# Autodesk Inventor assembly: tacho
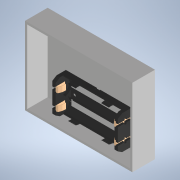
[picture p0: Inventor's stored thumbnail of the model, 180x180]
Saved by Autodesk Inventor 2022 (Build 260153000, 153)
## iProperties
Created: 2024-07-12
Part Number: tacho
Document SubType Name: Assembly
Designer: Капустяник Андрей
Author: Капустяник Андрей
## Documents named in this file (5)
- C:\Users\akapu\OneDrive\Документы\Git\camp2024\tacho_case\tacho.iam
- C:\Users\akapu\OneDrive\Документы\Git\camp2024\tacho_case\tacho_base.ipt
- C:\Users\akapu\OneDrive\Документы\Git\camp2024\tacho_case\WEH000802ALPP5N00000.ipt
- C:\Users\akapu\OneDrive\Документы\Git\camp2024\tacho_case\Hold_18650-2p_smd.ipt
- C:\Users\akapu\OneDrive\Документы\Git\camp2024\tacho_case\tacho_board.ipt
## Components (4 placed, 4 different names)
1. tacho_base:1 — Совмещение:3, Совмещение:4, Заподлицо:1, Совмещение:5, Совмещение:6
2. WEH000802ALPP5N00000:1 — Совмещение:2, Заподлицо:1, Совмещение:5, Совмещение:6
3. Hold_18650-2p_smd:1 — Совмещение:1, Совмещение:7
4. tacho_board:1 — Совмещение:1, Совмещение:2, Совмещение:3, Совмещение:4, Совмещение:7
## Relationships (8: Mate 7, Flush 1)
- Совмещение:1 [Mate]: Hold_18650-2p_smd:1 ↔ tacho_board:1
- Совмещение:2 [Mate] (2.54 mm): WEH000802ALPP5N00000:1 ↔ tacho_board:1
- Совмещение:3 [Mate]: tacho_base:1 ↔ tacho_board:1
- Совмещение:4 [Mate]: tacho_base:1 ↔ tacho_board:1
- Заподлицо:1 [Flush] (2 mm): tacho_base:1 ↔ WEH000802ALPP5N00000:1
- Совмещение:5 [Mate]: tacho_base:1 ↔ WEH000802ALPP5N00000:1
- Совмещение:6 [Mate]: tacho_base:1 ↔ WEH000802ALPP5N00000:1
- Совмещение:7 [Mate]: Hold_18650-2p_smd:1 ↔ tacho_board:1
